# Autodesk Inventor assembly: z-axis_assembly
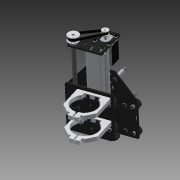
[picture p0: Inventor's stored thumbnail of the model, 180x180]
Saved by Autodesk Inventor 2014 (Build 180170000, 170)
## iProperties
Created: 2013-03-06
Part Number: z-axis_assembly
Document SubType Name: Assembly
Designer: Edward
Mass: 1567.3 g
Surface Area: 2632.04 cm^2
Volume: 388.503 cm^3
Density: 4.03421 g/cm^3
Author: Edward
## Documents named in this file (23)
- C:\Users\Edward\Desktop\Shapeoko_2.0_collection\Shapeoko_formed\Workgroups\Workgroup\z-axis_assembly.iam
- C:\Users\Edward\Desktop\Shapeoko_2.0_collection\Shapeoko_formed\Workgroups\Workgroup\z-belt.ipt
- C:\Users\Edward\Desktop\Shapeoko_2.0_collection\Shapeoko_formed\Workgroups\Workgroup\SM-E01.ipt
- C:\Users\Edward\Desktop\Shapeoko_2.0_collection\Shapeoko_formed\Workgroups\Workgroup\S2_MS200.ipt
- C:\Users\Edward\Desktop\Shapeoko_2.0_collection\Shapeoko_formed\Workgroups\Workgroup\S2_zplate-assembly.iam
- C:\Users\Edward\Desktop\Shapeoko_2.0_collection\Shapeoko_formed\Workgroups\Workgroup\SM-M08.ipt
- C:\Users\Edward\Desktop\Shapeoko_2.0_collection\Shapeoko_formed\Workgroups\Workgroup\z_mount_plate.ipt
- C:\Users\Edward\Desktop\Shapeoko_2.0_collection\Shapeoko_formed\Workgroups\Workgroup\7804K145.ipt
- C:\Users\Edward\Desktop\Shapeoko_2.0_collection\Shapeoko_formed\Workgroups\Workgroup\S2_zrod.ipt
- C:\Users\Edward\Desktop\Shapeoko_2.0_collection\Shapeoko_formed\Workgroups\Workgroup\DW660_Mount.ipt
- C:\Users\Edward\Desktop\Shapeoko_2.0_collection\Shapeoko_formed\Workgroups\Workgroup\SM-H03.ipt
- C:\Users\Edward\Desktop\Shapeoko_2.0_collection\Shapeoko_formed\Workgroups\Workgroup\SM-H04.ipt
- C:\Users\Edward\Desktop\Shapeoko_2.0_collection\Shapeoko_formed\Workgroups\Workgroup\91290A113.ipt
- C:\Users\Edward\Desktop\Shapeoko_2.0_collection\Shapeoko_formed\Workgroups\Workgroup\91166A210.ipt
- C:\Users\Edward\Desktop\Shapeoko_2.0_collection\Shapeoko_formed\Workgroups\Workgroup\plate_assembly.iam
- C:\Users\Edward\Desktop\Shapeoko_2.0_collection\Shapeoko_formed\Workgroups\Workgroup\91239A232.ipt
- C:\Users\Edward\Desktop\Shapeoko_2.0_collection\Shapeoko_formed\Workgroups\Workgroup\91239A228.ipt
- C:\Users\Edward\Desktop\Shapeoko_2.0_collection\Shapeoko_formed\Workgroups\Workgroup\z_screw_bottom_mount.ipt
- C:\Users\Edward\Desktop\Shapeoko_2.0_collection\Shapeoko_formed\Workgroups\Workgroup\a_6a51-020df0606.ipt
- C:\Users\Edward\Desktop\Shapeoko_2.0_collection\Shapeoko_formed\Workgroups\Workgroup\a_6a51-036df0908.ipt
- C:\Users\Edward\Desktop\Shapeoko_2.0_collection\Shapeoko_formed\Workgroups\Workgroup\HNKK55.ipt
- C:\Users\Edward\Desktop\Shapeoko_2.0_collection\Shapeoko_formed\Workgroups\Workgroup\#AS38-12-80.ipt
- C:\Users\Edward\Desktop\Shapeoko_2.0_collection\Shapeoko_formed\Workgroups\Workgroup\91290A260.ipt
## Components (93 placed, 22 different names)
1. z-belt:1 — Mate:15
2. SM-E01:1 — Insert:5, Insert:15, Mate:11, Mate:15, Angle:1
3. S2_MS200:1 — Mate:2, Flush:3, Mate:3, Flush:7, Insert:12, Insert:13, Insert:30, Insert:31, Mate:10, Flush:11, Flush:12
4. S2_zplate-assembly:1 [sub-assembly] — Mate:3, Mate:7, Flush:5, Flush:7, Insert:6, Insert:7, Insert:8, Insert:9, Insert:26, Insert:27, Insert:42, Insert:43, Insert:51, Mate:14, Insert:52, Insert:53, Insert:54, Insert:55
5. SM-M08:1 — Mate:6, Mate:7, Flush:5, Insert:34, Insert:35
6. z_mount_plate:1 — Mate:2, Flush:3, Insert:1, Insert:5, Angle:1
7. 7804K145:1 — Insert:1, Mate:12
8. S2_zrod:1 — Insert:3, Mate:6, Mate:12, Mate:13
9. 7804K145:2 — Insert:3, Insert:48
10. DW660_Mount:1 — Insert:6, Insert:7, Insert:22, Insert:23, Insert:54, Insert:55
11. DW660_Mount:2 — Insert:8, Insert:9, Insert:38, Insert:39
12. 91239A232:1 — Insert:45
13. 91239A232:2 — Insert:44
14. SM-H03:1 — Insert:13, Insert:44
15. SM-H04:1 — Insert:25
16. SM-H03:2 — Insert:12, Insert:45
17. SM-H04:2 — Insert:24
18. 91239A232:3 — Insert:57
19. SM-H03:5 — Insert:23, Insert:57
20. 91239A232:4 — Insert:56
21. SM-H03:6 — Insert:22, Insert:56
22. SM-H03:7 — Insert:25, Insert:26, Insert:53
23. SM-H03:8 — Insert:24, Insert:27, Insert:52
24. SM-H03:9 — Insert:30, Insert:46
25. 91239A232:5 — Insert:46
26. 91239A232:6 — Insert:47
27. SM-H03:10 — Insert:31, Insert:47
28. 91239A228:1
29. SM-H03:11 — Insert:34
30. 91239A228:2
31. SM-H03:12 — Insert:35
32. 91239A232:7 — Insert:50
33. SM-H03:13 — Insert:38, Insert:50, Mate:14
34. 91239A232:8 — Insert:49
35. SM-H03:14 — Insert:39, Insert:49
36. SM-H03:15 — Insert:41, Insert:43, Insert:51
37. SM-H04:3 — Insert:41
38. SM-H03:16 — Insert:40, Insert:42
39. SM-H04:4 — Insert:40
40. plate_assembly:1 [sub-assembly] — Mate:10, Flush:11, Mate:16, Mate:17, Mate:18, Mate:19, Insert:66, Insert:67, Insert:68, Insert:69, Insert:70, Insert:71, Insert:72, Insert:73, Insert:74, Insert:75, Insert:76, Insert:77
41. z_screw_bottom_mount:1 — Flush:12, Insert:48
42. a_6a51-020df0606:1 — Mate:11, Flush:14
43. a_6a51-036df0908:1 — Mate:13, Flush:14
44. 91239A228:3 — Insert:58
45. 91239A228:4 — Insert:59
46. 91239A228:5 — Insert:60
47. 91239A228:6 — Insert:61
48. SM-H03:17 — Insert:58, Insert:65, Mate:17
49. SM-H03:18 — Insert:59, Insert:64, Mate:16
50. SM-H03:19 — Insert:60, Insert:63, Mate:19
51. SM-H03:20 — Insert:61, Insert:62, Mate:18
52. HNKK55:1 — Insert:65
53. HNKK55:2 — Insert:64
54. HNKK55:3 — Insert:63
55. HNKK55:4 — Insert:62
56. #AS38-12-80:1 — Insert:66, Insert:83
57. #AS38-12-80:2 — Insert:69, Insert:79
58. #AS38-12-80:3 — Insert:68, Insert:81
59. #AS38-12-80:4 — Insert:71, Insert:87
60. #AS38-12-80:5 — Insert:67, Insert:85
61. #AS38-12-80:6 — Insert:70, Insert:89
62. 91290A260:1 — Insert:72, Insert:90
63. 91290A260:2 — Insert:73, Insert:91
64. 91290A260:3 — Insert:74, Insert:92
65. 91290A260:4 — Insert:75, Insert:93
66. 91290A260:5 — Insert:76, Insert:94
67. 91290A260:6 — Insert:77, Insert:95
68. SM-H04:5 — Insert:82
69. SM-H03:21 — Insert:82, Insert:83
70. SM-H04:6 — Insert:80
71. SM-H03:22 — Insert:80, Insert:81
72. SM-H04:7 — Insert:78
73. SM-H03:23 — Insert:78, Insert:79
74. SM-H04:8 — Insert:84
75. SM-H03:24 — Insert:84, Insert:85
76. SM-H04:9 — Insert:86
77. SM-H03:25 — Insert:86, Insert:87
78. SM-H04:10 — Insert:88
79. SM-H03:26 — Insert:88, Insert:89
80. SM-H03:27 — Insert:90
81. SM-H03:28 — Insert:91
82. SM-H03:29 — Insert:92
83. SM-H03:30 — Insert:93
84. SM-H03:31 — Insert:94
85. SM-H03:32 — Insert:95
86. 91166A210:1 — Insert:14, Insert:15
87. 91290A113:1 — Insert:14
88. 91166A210:2
89. 91290A113:2
90. 91166A210:3
91. 91290A113:3
92. 91166A210:4
93. 91290A113:4
## Component patterns: (4 elements, first: 91166A210:1 + 91290A113:1)
## Relationships (110: Insert 89, Mate 14, Flush 6, Angle 1)
- Mate:2: S2_MS200:1 ↔ z_mount_plate:1
- Flush:3: S2_MS200:1 ↔ z_mount_plate:1
- Mate:3 (6.37 mm): S2_MS200:1 ↔ S2_zplate-assembly:1
- Insert:1: z_mount_plate:1 ↔ 7804K145:1
- Insert:3: S2_zrod:1 ↔ 7804K145:2
- Insert:5: SM-E01:1 ↔ z_mount_plate:1
- Mate:6: SM-M08:1 ↔ S2_zrod:1
- Mate:7: S2_zplate-assembly:1 ↔ SM-M08:1
- Flush:5 (45 mm): S2_zplate-assembly:1 ↔ SM-M08:1
- Flush:7 (-21.752 mm): S2_MS200:1 ↔ S2_zplate-assembly:1
- Insert:6: S2_zplate-assembly:1 ↔ DW660_Mount:1
- Insert:7: S2_zplate-assembly:1 ↔ DW660_Mount:1
- Insert:8: S2_zplate-assembly:1 ↔ DW660_Mount:2
- Insert:9: S2_zplate-assembly:1 ↔ DW660_Mount:2
- [Insert]: 91239A232:2 ↔ SM-H03:1
- [Insert]: 91239A232:1 ↔ SM-H03:2
- Insert:12 (3.4163 mm): S2_MS200:1 ↔ SM-H03:2
- Insert:13 (3.4163 mm): S2_MS200:1 ↔ SM-H03:1
- Insert:14: 91166A210:1 ↔ 91290A113:1
- Insert:15 (3.4163 mm): SM-E01:1 ↔ 91166A210:1
- [Insert]: 91239A232:3 ↔ SM-H03:5
- [Insert]: 91239A232:4 ↔ SM-H03:6
- Insert:22: DW660_Mount:1 ↔ SM-H03:6
- Insert:23: DW660_Mount:1 ↔ SM-H03:5
- Insert:24: SM-H04:2 ↔ SM-H03:8
- Insert:25: SM-H04:1 ↔ SM-H03:7
- Insert:26: S2_zplate-assembly:1 ↔ SM-H03:7
- Insert:27: S2_zplate-assembly:1 ↔ SM-H03:8
- [Insert]: 91239A232:6 ↔ SM-H03:10
- [Insert]: SM-H03:9 ↔ 91239A232:5
- Insert:30 (3.4163 mm): S2_MS200:1 ↔ SM-H03:9
- Insert:31 (3.4163 mm): S2_MS200:1 ↔ SM-H03:10
- [Insert]: 91239A228:2 ↔ SM-H03:12
- [Insert]: 91239A228:1 ↔ SM-H03:11
- Insert:34 (3.4163 mm): SM-M08:1 ↔ SM-H03:11
- Insert:35 (3.4163 mm): SM-M08:1 ↔ SM-H03:12
- [Insert]: 91239A232:7 ↔ SM-H03:13
- [Insert]: 91239A232:8 ↔ SM-H03:14
- Insert:38: DW660_Mount:2 ↔ SM-H03:13
- Insert:39: DW660_Mount:2 ↔ SM-H03:14
- Insert:40: SM-H03:16 ↔ SM-H04:4
- Insert:41: SM-H03:15 ↔ SM-H04:3
- Insert:42: S2_zplate-assembly:1 ↔ SM-H03:16
- Insert:43: S2_zplate-assembly:1 ↔ SM-H03:15
- Mate:10: S2_MS200:1 ↔ plate_assembly:1
- Flush:11 (-60 mm): S2_MS200:1 ↔ plate_assembly:1
- Flush:12: S2_MS200:1 ↔ z_screw_bottom_mount:1
- Insert:44: 91239A232:2 ↔ SM-H03:1
- Insert:45: 91239A232:1 ↔ SM-H03:2
- Mate:11: SM-E01:1 ↔ a_6a51-020df0606:1
- Insert:46: SM-H03:9 ↔ 91239A232:5
- Insert:47: 91239A232:6 ↔ SM-H03:10
- Insert:48: 7804K145:2 ↔ z_screw_bottom_mount:1
- Mate:12: 7804K145:1 ↔ S2_zrod:1
- Mate:13: S2_zrod:1 ↔ a_6a51-036df0908:1
- Flush:14: a_6a51-020df0606:1 ↔ a_6a51-036df0908:1
- Insert:49: 91239A232:8 ↔ SM-H03:14
- Insert:50: 91239A232:7 ↔ SM-H03:13
- Insert:51: S2_zplate-assembly:1 ↔ SM-H03:15
- Mate:14: S2_zplate-assembly:1 ↔ SM-H03:13
- Insert:52: S2_zplate-assembly:1 ↔ SM-H03:8
- Insert:53: S2_zplate-assembly:1 ↔ SM-H03:7
- Insert:54: S2_zplate-assembly:1 ↔ DW660_Mount:1
- Insert:55: S2_zplate-assembly:1 ↔ DW660_Mount:1
- Insert:56: 91239A232:4 ↔ SM-H03:6
- Insert:57: 91239A232:3 ↔ SM-H03:5
- Mate:15: z-belt:1 ↔ SM-E01:1
- Angle:1 (0 deg): SM-E01:1 ↔ z_mount_plate:1
- Insert:58: 91239A228:3 ↔ SM-H03:17
- Insert:59: 91239A228:4 ↔ SM-H03:18
- Insert:60: 91239A228:5 ↔ SM-H03:19
- Insert:61: 91239A228:6 ↔ SM-H03:20
- Insert:62 (7 mm): SM-H03:20 ↔ HNKK55:4
- Insert:63 (7 mm): SM-H03:19 ↔ HNKK55:3
- Insert:64 (7 mm): SM-H03:18 ↔ HNKK55:2
- Insert:65 (7 mm): SM-H03:17 ↔ HNKK55:1
- Mate:16: plate_assembly:1 ↔ SM-H03:18
- Mate:17: plate_assembly:1 ↔ SM-H03:17
- Mate:18: plate_assembly:1 ↔ SM-H03:20
- Mate:19: plate_assembly:1 ↔ SM-H03:19
- Insert:66: plate_assembly:1 ↔ #AS38-12-80:1
- Insert:67: plate_assembly:1 ↔ #AS38-12-80:5
- Insert:68: plate_assembly:1 ↔ #AS38-12-80:3
- Insert:69: plate_assembly:1 ↔ #AS38-12-80:2
- Insert:70: plate_assembly:1 ↔ #AS38-12-80:6
- Insert:71: plate_assembly:1 ↔ #AS38-12-80:4
- Insert:72: plate_assembly:1 ↔ 91290A260:1
- Insert:73: plate_assembly:1 ↔ 91290A260:2
- Insert:74: plate_assembly:1 ↔ 91290A260:3
- Insert:75: plate_assembly:1 ↔ 91290A260:4
- Insert:76: plate_assembly:1 ↔ 91290A260:5
- Insert:77: plate_assembly:1 ↔ 91290A260:6
- Insert:78: SM-H04:7 ↔ SM-H03:23
- Insert:79 (3.5 mm): #AS38-12-80:2 ↔ SM-H03:23
- Insert:80: SM-H04:6 ↔ SM-H03:22
- Insert:81 (3.5 mm): #AS38-12-80:3 ↔ SM-H03:22
- Insert:82: SM-H04:5 ↔ SM-H03:21
- Insert:83 (3.5 mm): #AS38-12-80:1 ↔ SM-H03:21
- Insert:84: SM-H04:8 ↔ SM-H03:24
- Insert:85 (3.5 mm): #AS38-12-80:5 ↔ SM-H03:24
- Insert:86: SM-H04:9 ↔ SM-H03:25
- Insert:87 (3.5 mm): #AS38-12-80:4 ↔ SM-H03:25
- Insert:88: SM-H04:10 ↔ SM-H03:26
- Insert:89 (3.5 mm): #AS38-12-80:6 ↔ SM-H03:26
- Insert:90: 91290A260:1 ↔ SM-H03:27
- Insert:91: 91290A260:2 ↔ SM-H03:28
- Insert:92: 91290A260:3 ↔ SM-H03:29
- Insert:93: 91290A260:4 ↔ SM-H03:30
- Insert:94: 91290A260:5 ↔ SM-H03:31
- Insert:95: 91290A260:6 ↔ SM-H03:32
